# Autodesk Inventor assembly: Knights Mobile platform design
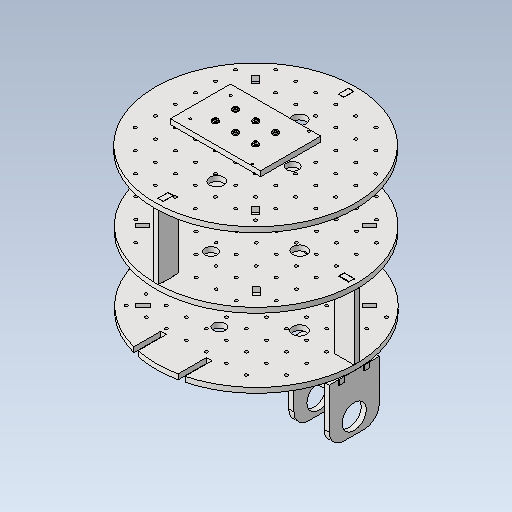
[picture p0: Inventor's stored thumbnail of the model, 512x512]
Saved by Autodesk Inventor 2025 (Build 290162000, 162)
## iProperties
Created: 2024-08-13
Part Number: Knights Mobile platform design
Document SubType Name: Assembly
Designer: PC
Author: PC
## Documents named in this file (8)
- C:\Users\HP\Downloads\Compressed\KNIGHTS mobile platform CAD files\Knights Mobile platform design.iam
- C:\Users\HP\Downloads\Compressed\KNIGHTS mobile platform CAD files\baseplate.ipt
- C:\Users\HP\Downloads\Compressed\KNIGHTS mobile platform CAD files\custom standoffs.ipt
- C:\Users\HP\Downloads\Compressed\KNIGHTS mobile platform CAD files\midPlate.ipt
- C:\Users\HP\Downloads\Compressed\KNIGHTS mobile platform CAD files\Top plate.ipt
- C:\Users\HP\Downloads\Compressed\KNIGHTS mobile platform CAD files\lidar mounting plate.ipt
- C:\Users\HP\Documents\Inventor\Content Center Files\R2025\en-US\IS 7483\IS 7483 - M3 x 8.ipt
- C:\Users\HP\Downloads\Compressed\KNIGHTS mobile platform CAD files\motorchassisholder2Ass.iam
## Components (16 placed, 7 different names)
1. baseplate:1 — Mate:1, Mate:2, Flush:1, Flush:2, Flush:3, Mate:3, Flush:4, Flush:5, Mate:4, Mate:10, Mate:11, Angle:1
2. custom standoffs:1 — Flush:2, Flush:3, Mate:3, Flush:6, Flush:7, Mate:5, Flush:16
3. custom standoffs:2 — Flush:4, Flush:5, Mate:4, Flush:15, Flush:17
4. midPlate:1 — Flush:6, Flush:7, Mate:5, Flush:8, Flush:9, Mate:6, Flush:10, Flush:11, Mate:7
5. custom standoffs:3 — Flush:8, Flush:9, Mate:6, Flush:12, Flush:13, Mate:8
6. custom standoffs:4 — Flush:10, Flush:11, Mate:7
7. Top plate:1 — Flush:12, Flush:13, Mate:8, Insert:7, Insert:8
8. lidar mounting plate:1 — Insert:1, Insert:2, Insert:3, Insert:4, Insert:5, Insert:6
9. IS 7483 M3 x 8:1 — Insert:1
10. IS 7483 M3 x 8:2 — Insert:4, Insert:7
11. IS 7483 M3 x 8:3 — Insert:2
12. IS 7483 M3 x 8:4 — Insert:5
13. IS 7483 M3 x 8:5 — Insert:3, Insert:8
14. IS 7483 M3 x 8:6 — Insert:6
15. motorchassisholder2Ass:1 [sub-assembly] — Mate:10, Flush:14, Flush:16
16. motorchassisholder2Ass:2 [sub-assembly] — Flush:14, Mate:11, Angle:1, Flush:15, Flush:17
## Relationships (36: Flush 17, Mate 10, Insert 8, Angle 1)
- Mate:1: baseplate:1
- Mate:2: baseplate:1
- Flush:1: baseplate:1
- Flush:2 (-0.3 mm): baseplate:1 ↔ custom standoffs:1
- Flush:3 (-10 mm): baseplate:1 ↔ custom standoffs:1
- Mate:3: baseplate:1 ↔ custom standoffs:1
- Flush:4 (69.6 mm): baseplate:1 ↔ custom standoffs:2
- Flush:5 (10 mm): baseplate:1 ↔ custom standoffs:2
- Mate:4: baseplate:1 ↔ custom standoffs:2
- Flush:6 (-190 mm): custom standoffs:1 ↔ midPlate:1
- Flush:7 (-0.3 mm): custom standoffs:1 ↔ midPlate:1
- Mate:5: custom standoffs:1 ↔ midPlate:1
- Flush:8 (-0.3 mm): midPlate:1 ↔ custom standoffs:3
- Flush:9 (-5.1 mm): midPlate:1 ↔ custom standoffs:3
- Mate:6: midPlate:1 ↔ custom standoffs:3
- Flush:10 (-0.3 mm): midPlate:1 ↔ custom standoffs:4
- Flush:11 (-10 mm): midPlate:1 ↔ custom standoffs:4
- Mate:7: midPlate:1 ↔ custom standoffs:4
- Flush:12 (5.1 mm): custom standoffs:3 ↔ Top plate:1
- Flush:13 (0.3 mm): custom standoffs:3 ↔ Top plate:1
- Mate:8: custom standoffs:3 ↔ Top plate:1
- Insert:1: lidar mounting plate:1 ↔ IS 7483 M3 x 8:1
- Insert:2: lidar mounting plate:1 ↔ IS 7483 M3 x 8:3
- Insert:3: lidar mounting plate:1 ↔ IS 7483 M3 x 8:5
- Insert:4: lidar mounting plate:1 ↔ IS 7483 M3 x 8:2
- Insert:5: lidar mounting plate:1 ↔ IS 7483 M3 x 8:4
- Insert:6: lidar mounting plate:1 ↔ IS 7483 M3 x 8:6
- Insert:7 (-2.9 mm): Top plate:1 ↔ IS 7483 M3 x 8:2
- Insert:8 (-2.9 mm): Top plate:1 ↔ IS 7483 M3 x 8:5
- Mate:10: baseplate:1 ↔ motorchassisholder2Ass:1
- Flush:14: motorchassisholder2Ass:1 ↔ motorchassisholder2Ass:2
- Mate:11: baseplate:1 ↔ motorchassisholder2Ass:2
- Angle:1 (0 deg): baseplate:1 ↔ motorchassisholder2Ass:2
- Flush:15: custom standoffs:2 ↔ motorchassisholder2Ass:2
- Flush:16: custom standoffs:1 ↔ motorchassisholder2Ass:1
- Flush:17 (20 mm): custom standoffs:2 ↔ motorchassisholder2Ass:2
